# Autodesk Inventor assembly: R-T v4
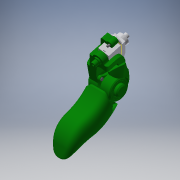
[picture p0: Inventor's stored thumbnail of the model, 180x180]
Saved by Autodesk Inventor 2018.2 (Build 222227000, 227)
## iProperties
Created: 2017-09-22
Part Number: R-T v4
Material: 一般
Document SubType Name: Assembly
Designer: sktom
Author: sktom
## Documents named in this file (11)
- D:\CloudStrage\OneDrive\CADMech\HbSizeMMech\UnitHand\Unit_MR-H\Unit_MR-T\Unit_MR-T.iam
- D:\CloudStrage\OneDrive\CADMech\HbSizeMMech\UnitHand\Unit_MR-H\Unit_MR-T\MR-T-03.ipt
- D:\CloudStrage\OneDrive\CADMech\HbSizeMMech\UnitHand\Unit_MR-H\Unit_MR-T\MR-T-02.ipt
- D:\CloudStrage\OneDrive\CADMech\HbSizeMMech\UnitHand\Unit_MR-H\Unit_MR-T\MR-T-01.ipt
- D:\CloudStrage\OneDrive\CADMech\HbSizeMMech\UnitHand\Unit_MR-H\Unit_MR-T\MR-T-04.ipt
- D:\CloudStrage\OneDrive\CADMech\HbSizeMMech\UnitHand\Unit_MR-H\Unit_MR-T\MR-T-05.ipt
- D:\CloudStrage\OneDrive\CADMech\HbSizeMMech\UnitHand\Unit_MR-H\Unit_MR-T\MR-T-06.ipt
- D:\CloudStrage\OneDrive\CADMech\HbSizeMMech\UnitHand\Unit_MR-H\Unit_MR-T\Parts_Servo_HK282A.ipt
- D:\CloudStrage\OneDrive\CADMech\HbSizeMMech\UnitHand\Unit_MR-H\Unit_MR-T\Parts_Screw_M1.7_L8.ipt
- D:\CloudStrage\OneDrive\CADMech\HbSizeMMech\UnitHand\Unit_MR-H\Unit_MR-T\Parts_CoilSpring_CP 0.6-5.5-8.ipt
- D:\CloudStrage\OneDrive\CADMech\HbSizeMMech\UnitHand\Unit_MR-H\Unit_MR-T\Parts_FlatScrew_M2_L6.ipt
## Components (14 placed, 10 different names)
1. MR-T-01 — 角度:1, 挿入:5
2. MR-T-02 — 回転:3, 角度:1
3. MR-T-03 — 回転:3, リジッド:1, 挿入:6, 挿入:7
4. MR-T-04 — リジッド:1
5. MR-T-05 — 円柱状:2, 挿入:3, 挿入:4
6. MR-T-06 — 円柱状:2, 挿入:2
7. Parts_CoilSpring_CP 0.6-5.5-8:1 — 挿入:6
8. Parts_Servo_HK282A:1 — 挿入:1
9. Parts_Screw_M1.7_L8:1 — 挿入:1
10. Parts_Screw_M1.7_L8:2 — 挿入:2
11. Parts_Screw_M1.7_L8:3 — 挿入:3
12. Parts_Screw_M1.7_L8:4 — 挿入:4
13. Parts_Screw_M1.7_L8:5 — 挿入:5
14. Parts_FlatScrew_M2_L6:1 — 挿入:7
## Relationships (11: Insert 7, RevoluteJoint 1, Angle 1, WeldJoint 1, CylindricalJoint 1)
- 回転:3 [RevoluteJoint] (-0.3 mm): MR-T-02 ↔ MR-T-03
- 角度:1 [Angle] (180 deg): MR-T-01 ↔ MR-T-02
- リジッド:1 [WeldJoint] (3 mm): MR-T-03 ↔ MR-T-04
- 円柱状:2 [CylindricalJoint]: MR-T-05 ↔ MR-T-06
- 挿入:1 [Insert]: Parts_Servo_HK282A:1 ↔ Parts_Screw_M1.7_L8:1
- 挿入:2 [Insert]: MR-T-06 ↔ Parts_Screw_M1.7_L8:2
- 挿入:3 [Insert]: MR-T-05 ↔ Parts_Screw_M1.7_L8:3
- 挿入:4 [Insert]: MR-T-05 ↔ Parts_Screw_M1.7_L8:4
- 挿入:5 [Insert]: MR-T-01 ↔ Parts_Screw_M1.7_L8:5
- 挿入:6 [Insert]: MR-T-03 ↔ Parts_CoilSpring_CP 0.6-5.5-8:1
- 挿入:7 [Insert]: MR-T-03 ↔ Parts_FlatScrew_M2_L6:1
